# Autodesk Inventor assembly: InsulatorWall
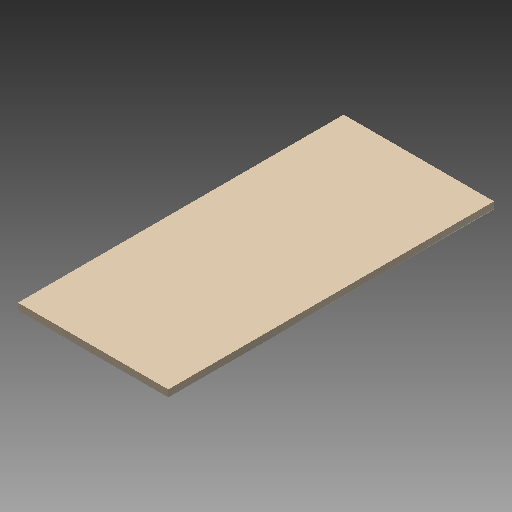
[picture p0: Inventor's stored thumbnail of the model, 512x512]
Saved by Autodesk Inventor 2017 (Build 210142000, 142)
## iProperties
Created: 2016-12-13
Part Number: InsulatorWall
Document SubType Name: Assembly
Designer: umr
Author: umr
## Documents named in this file (3)
- D:\SeniorProject\Models2\Case\WideWall.iam
- D:\SeniorProject\Models2\Case\ReflectorWallWide.ipt
- D:\SeniorProject\Models2\Case\InsulatorWallWide.ipt
## Components (2 placed, 2 different names)
1. ReflectorWallWide:1 — Mate:1, Flush:1, Flush:2
2. InsulatorWallWide:1 — Mate:1, Flush:1, Flush:2
## Relationships (3: Flush 2, Mate 1)
- Mate:1: ReflectorWallWide:1 ↔ InsulatorWallWide:1
- Flush:1: ReflectorWallWide:1 ↔ InsulatorWallWide:1
- Flush:2: ReflectorWallWide:1 ↔ InsulatorWallWide:1
